# Autodesk Inventor assembly: upper_arm
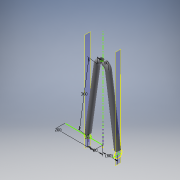
[picture p0: Inventor's stored thumbnail of the model, 180x180]
Saved by Autodesk Inventor 2016 SP1 (Build 200210100, 210)
## iProperties
Created: 2016-06-15
Part Number: upper_arm
Document SubType Name: Assembly
Designer: asvsf
Author: asvsf
## Documents named in this file (3)
- C:\Project\Buggy\Suspension\upper_arm.iam
- C:\Project\Buggy\Suspension\upper_arm_001.ipt
- C:\Project\Buggy\Suspension\upper_arm_005.ipt
## Components (2 placed, 2 different names)
1. upper_arm_001:1 — Mate:21, Mate:26
2. upper_arm_005:1 — Mate:26
## Relationships (2: Mate 2)
- Mate:21: upper_arm_001:1
- Mate:26: upper_arm_001:1 ↔ upper_arm_005:1
